# Autodesk Inventor assembly: Skirt Side [B]
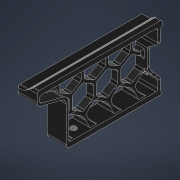
[picture p0: Inventor's stored thumbnail of the model, 180x180]
Saved by Autodesk Inventor 2022.2 (Build 262287010, 287A)
## iProperties
Created: 2022-03-13
Part Number: Skirt Side [B]
Document SubType Name: Assembly
Designer: sleib
Author: sleib
## Documents named in this file (3)
- C:\Users\sleib\Projekte\Voron-2\CAD\Inventor\Skirt Side [B].iam
- C:\Users\sleib\Projekte\Voron-2\CAD\Inventor\Skirt Side (350mm) [B].ipt
- C:\Users\sleib\Projekte\Voron-2\CAD\Inventor\M3x8 SHCS.ipt
## Components (2 placed, 2 different names)
1. Skirt Side (350mm) [B]:1 — Passend:1, Passend:2
2. M3x8 SHCS:1 — Passend:1, Passend:2
## Relationships (2: Mate 2)
- Passend:1 [Mate]: Skirt Side (350mm) [B]:1 ↔ M3x8 SHCS:1
- Passend:2 [Mate]: Skirt Side (350mm) [B]:1 ↔ M3x8 SHCS:1
